# Autodesk Inventor assembly: mount_battery
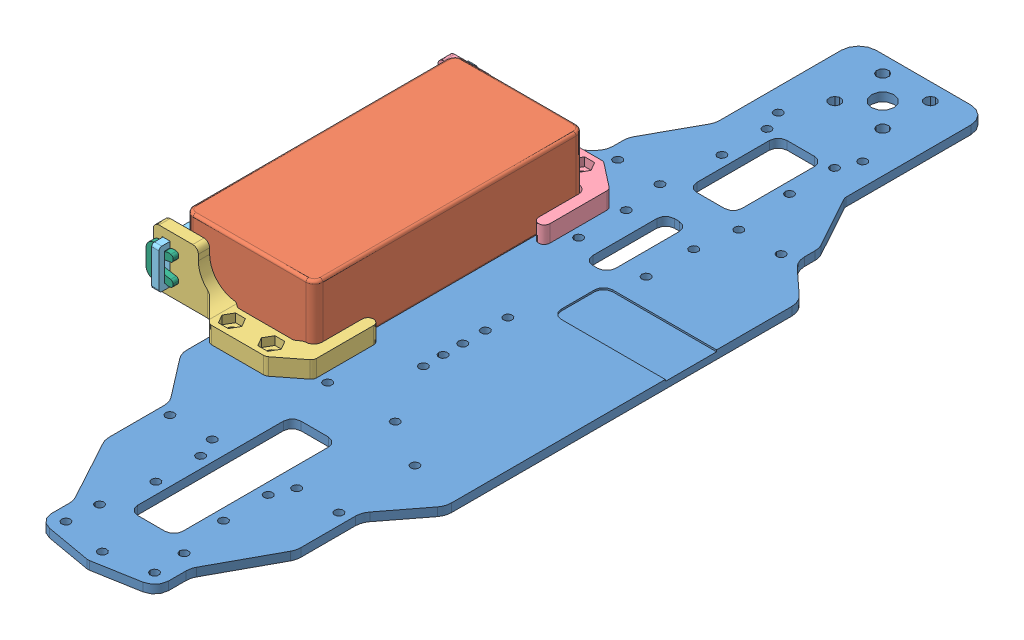
[picture p0: shaded view drawn from the shape stored in the file]
Saved by Autodesk Inventor 2021 (Build 250183000, 183)
## iProperties
Created: 2021-01-30
Part Number: mount_battery
Document SubType Name: Assembly
Designer: User
Author: User
## Documents named in this file (7)
- D:\SynologyDrive\tcodev\tco-cad\mount_battery\mount_battery.iam
- D:\SynologyDrive\tcodev\tco-cad\chassis_short\base_short.ipt
- D:\SynologyDrive\tcodev\tco-cad\common\battery.ipt
- D:\SynologyDrive\tcodev\tco-cad\mount_battery\mount_battery.ipt
- D:\SynologyDrive\tcodev\tco-cad\mount_battery\mount_battery_mirrored.ipt
- D:\SynologyDrive\tcodev\tco-cad\mount_battery\mount_battery_fastener.ipt
- D:\SynologyDrive\tcodev\tco-cad\mount_battery\fastener_lock.ipt
## Components (7 placed, 6 different names)
1. base_short:1 — Mate:1, Flush:1, Mate:2, Rigid:1
2. battery:1 — Mate:1
3. mount_battery:1 — Flush:1
4. mount_battery_mirrored:1 — Mate:2, Mate:3, Rigid:1, Mate:4, Flush:2
5. mount_battery_fastener:1 — Mate:3, Mate:4, Flush:2, Mate:5, Mate:6, Mate:7
6. fastener_lock:1 — Mate:5, Flush:3
7. fastener_lock:2 — Mate:6, Mate:7, Flush:3
## Relationships (11: Mate 7, Flush 3, WeldJoint 1)
- Mate:1: base_short:1 ↔ battery:1
- Flush:1: base_short:1 ↔ mount_battery:1
- Mate:2: base_short:1 ↔ mount_battery_mirrored:1
- Mate:3: mount_battery_mirrored:1 ↔ mount_battery_fastener:1
- Rigid:1 [WeldJoint]: base_short:1 ↔ mount_battery_mirrored:1
- Mate:4: mount_battery_mirrored:1 ↔ mount_battery_fastener:1
- Flush:2: mount_battery_mirrored:1 ↔ mount_battery_fastener:1
- Mate:5: mount_battery_fastener:1 ↔ fastener_lock:1
- Mate:6: mount_battery_fastener:1 ↔ fastener_lock:2
- Mate:7 (0.2 mm): mount_battery_fastener:1 ↔ fastener_lock:2
- Flush:3: fastener_lock:1 ↔ fastener_lock:2
